# Autodesk Inventor assembly: SHOT_1_002_ShooterAssembly
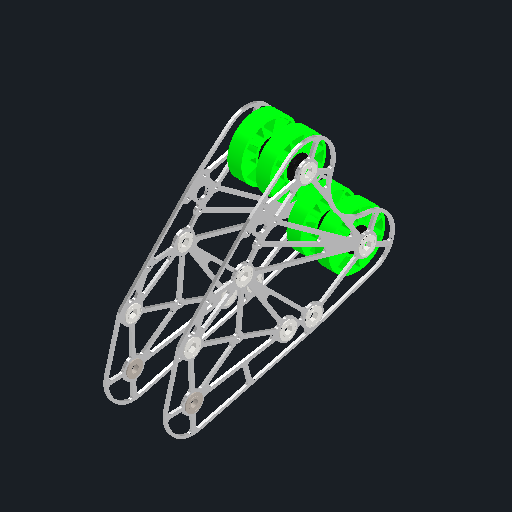
[picture p0: Inventor's stored thumbnail of the model, 512x512]
Saved by Autodesk Inventor 2024.2 (Build 282272000, 272)
## iProperties
Created: 2024-08-07
Part Number: SHOT_1_002_ShooterAssembly
Document SubType Name: Assembly
Designer: Kenji
Mass: 1474.99 g
Surface Area: 3908.93 cm^2
Volume: 710.058 cm^3
Density: 2.07728 g/cm^3
Author: Kenji
## Documents named in this file (5)
- C:\Users\bobsb\OneDrive\Documents\GitHub\1622-2024-Summer-CAD-A-Thon\Shooter\SHOT_1_002_ShooterAssembly.iam
- C:\Users\bobsb\OneDrive\Documents\GitHub\1622-2024-Summer-CAD-A-Thon\Shooter\SHOT_1_001_ShooterPlate.ipt
- C:\Users\bobsb\OneDrive\Documents\GitHub\1622-2024-Summer-CAD-A-Thon\COTS Library\Motion\Wheels\Compliant Wheels\4in compliant wheels\0.500in hex bore\COTS_am-3462_4indiameter_0.500inhexbore_durometer35A_CompliantWheel.ipt
- C:\Users\bobsb\OneDrive\Documents\GitHub\1622-2024-Summer-CAD-A-Thon\COTS Library\Motion\Bearings\COTS_WCP-0783_1.125ODHexBearing.ipt
- C:\Users\bobsb\OneDrive\Documents\GitHub\1622-2024-Summer-CAD-A-Thon\COTS Library\Motion\Bearings\COTS_WCP-0781_0.5ODCircularFlangedBearing.ipt
## Components (20 placed, 4 different names)
1. SHOT_1_001_ShooterPlate:1 — Mate:1, Mate:2, Mate:3, Mate:4, Mate:5, Mate:6, Mate:7, Mate:8, Mate:10, Mate:11, Mate:12, Mate:13, Mate:14, Mate:16, Mate:40, Mate:41, Mate:43
2. SHOT_1_001_ShooterPlate:2 — Mate:1, Mate:2, Mate:17, Mate:18, Mate:19, Mate:20, Mate:21, Mate:23, Mate:24, Mate:25, Mate:26, Mate:28, Mate:29, Mate:30, Mate:39, Mate:42, Mate:43, Mate:44, Mate:45
3. COTS_WCP-0783_1.125ODHexBearing:1 — Mate:17, Mate:30
4. COTS_WCP-0783_1.125ODHexBearing:2 — Mate:21, Mate:26
5. COTS_WCP-0783_1.125ODHexBearing:3 — Mate:18, Mate:24, Mate:36
6. COTS_WCP-0783_1.125ODHexBearing:4 — Mate:23, Mate:28
7. COTS_WCP-0783_1.125ODHexBearing:5 — Mate:7, Mate:14
8. COTS_WCP-0783_1.125ODHexBearing:6 — Mate:6, Mate:13
9. COTS_WCP-0783_1.125ODHexBearing:8 — Mate:8, Mate:16
10. COTS_WCP-0783_1.125ODHexBearing:9 — Mate:4, Mate:10
11. COTS_WCP-0783_1.125ODHexBearing:10 — Mate:3, Mate:11, Mate:31
12. COTS_WCP-0783_1.125ODHexBearing:11 — Mate:5, Mate:12
13. COTS_WCP-0783_1.125ODHexBearing:12 — Mate:20, Mate:29
14. COTS_WCP-0783_1.125ODHexBearing:13 — Mate:19, Mate:25
15. COTS_WCP-0781_0.5ODCircularFlangedBearing:1 — Mate:39, Mate:42
16. COTS_WCP-0781_0.5ODCircularFlangedBearing:2 — Mate:40, Mate:41
17. COTS_am-3462_4indiameter_0.500inhexbore_durometer35A_CompliantWheel:4 — Mate:36
18. COTS_am-3462_4indiameter_0.500inhexbore_durometer35A_CompliantWheel:1 — Mate:31
19. COTS_am-3462_4indiameter_0.500inhexbore_durometer35A_CompliantWheel:5 — Mate:45
20. COTS_am-3462_4indiameter_0.500inhexbore_durometer35A_CompliantWheel:6 — Mate:44
## Component patterns: (2 elements, first: COTS_am-3462_4indiameter_0.500inhexbore_durometer35A_CompliantWheel:4 + COTS_am-3462_4indiameter_0.500inhexbore_durometer35A_CompliantWheel:1)
## Relationships (35: Mate 35)
- Mate:1: SHOT_1_001_ShooterPlate:1 ↔ SHOT_1_001_ShooterPlate:2
- Mate:2: SHOT_1_001_ShooterPlate:1 ↔ SHOT_1_001_ShooterPlate:2
- Mate:3: SHOT_1_001_ShooterPlate:1 ↔ COTS_WCP-0783_1.125ODHexBearing:10
- Mate:4: SHOT_1_001_ShooterPlate:1 ↔ COTS_WCP-0783_1.125ODHexBearing:9
- Mate:5: SHOT_1_001_ShooterPlate:1 ↔ COTS_WCP-0783_1.125ODHexBearing:11
- Mate:6: SHOT_1_001_ShooterPlate:1 ↔ COTS_WCP-0783_1.125ODHexBearing:6
- Mate:7: SHOT_1_001_ShooterPlate:1 ↔ COTS_WCP-0783_1.125ODHexBearing:5
- Mate:8: SHOT_1_001_ShooterPlate:1 ↔ COTS_WCP-0783_1.125ODHexBearing:8
- Mate:10: SHOT_1_001_ShooterPlate:1 ↔ COTS_WCP-0783_1.125ODHexBearing:9
- Mate:11: SHOT_1_001_ShooterPlate:1 ↔ COTS_WCP-0783_1.125ODHexBearing:10
- Mate:12: SHOT_1_001_ShooterPlate:1 ↔ COTS_WCP-0783_1.125ODHexBearing:11
- Mate:13: SHOT_1_001_ShooterPlate:1 ↔ COTS_WCP-0783_1.125ODHexBearing:6
- Mate:14: SHOT_1_001_ShooterPlate:1 ↔ COTS_WCP-0783_1.125ODHexBearing:5
- Mate:16: SHOT_1_001_ShooterPlate:1 ↔ COTS_WCP-0783_1.125ODHexBearing:8
- Mate:17: SHOT_1_001_ShooterPlate:2 ↔ COTS_WCP-0783_1.125ODHexBearing:1
- Mate:18: SHOT_1_001_ShooterPlate:2 ↔ COTS_WCP-0783_1.125ODHexBearing:3
- Mate:19: SHOT_1_001_ShooterPlate:2 ↔ COTS_WCP-0783_1.125ODHexBearing:13
- Mate:20: SHOT_1_001_ShooterPlate:2 ↔ COTS_WCP-0783_1.125ODHexBearing:12
- Mate:21: SHOT_1_001_ShooterPlate:2 ↔ COTS_WCP-0783_1.125ODHexBearing:2
- Mate:23: SHOT_1_001_ShooterPlate:2 ↔ COTS_WCP-0783_1.125ODHexBearing:4
- Mate:24: SHOT_1_001_ShooterPlate:2 ↔ COTS_WCP-0783_1.125ODHexBearing:3
- Mate:25: SHOT_1_001_ShooterPlate:2 ↔ COTS_WCP-0783_1.125ODHexBearing:13
- Mate:26: SHOT_1_001_ShooterPlate:2 ↔ COTS_WCP-0783_1.125ODHexBearing:2
- Mate:28: SHOT_1_001_ShooterPlate:2 ↔ COTS_WCP-0783_1.125ODHexBearing:4
- Mate:29: SHOT_1_001_ShooterPlate:2 ↔ COTS_WCP-0783_1.125ODHexBearing:12
- Mate:30: SHOT_1_001_ShooterPlate:2 ↔ COTS_WCP-0783_1.125ODHexBearing:1
- Mate:31: COTS_WCP-0783_1.125ODHexBearing:10 ↔ COTS_am-3462_4indiameter_0.500inhexbore_durometer35A_CompliantWheel:1
- Mate:36: COTS_WCP-0783_1.125ODHexBearing:3 ↔ COTS_am-3462_4indiameter_0.500inhexbore_durometer35A_CompliantWheel:4
- Mate:39: SHOT_1_001_ShooterPlate:2 ↔ COTS_WCP-0781_0.5ODCircularFlangedBearing:1
- Mate:40: SHOT_1_001_ShooterPlate:1 ↔ COTS_WCP-0781_0.5ODCircularFlangedBearing:2
- Mate:41: SHOT_1_001_ShooterPlate:1 ↔ COTS_WCP-0781_0.5ODCircularFlangedBearing:2
- Mate:42: SHOT_1_001_ShooterPlate:2 ↔ COTS_WCP-0781_0.5ODCircularFlangedBearing:1
- Mate:43 (101.6 mm): SHOT_1_001_ShooterPlate:1 ↔ SHOT_1_001_ShooterPlate:2
- Mate:44 (12.7 mm): SHOT_1_001_ShooterPlate:2 ↔ COTS_am-3462_4indiameter_0.500inhexbore_durometer35A_CompliantWheel:6
- Mate:45 (12.7 mm): SHOT_1_001_ShooterPlate:2 ↔ COTS_am-3462_4indiameter_0.500inhexbore_durometer35A_CompliantWheel:5
